# Autodesk Inventor assembly: MaquinaDeCorte
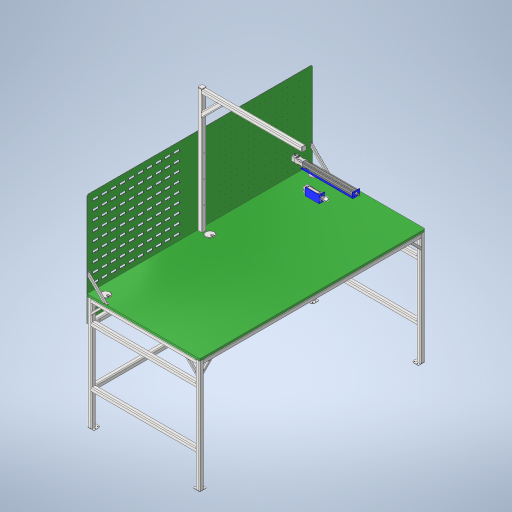
[picture p0: Inventor's stored thumbnail of the model, 512x512]
Saved by Autodesk Inventor 2023 (Build 270158000, 158)
## iProperties
Created: 2023-04-07
Part Number: MaquinaDeCorte
Document SubType Name: Assembly
Designer: Lenovo
Author: Lenovo
## Documents named in this file (6)
- D:\Esdek\Gemelo Digital\Corte de Tubos\MaquinaDeCorte.iam
- D:\Esdek\Gemelo Digital\Corte de Tubos\CADimportados\PistónElectromecánico\1470706 EPCO-25-300-3P-ST-E---(0).iam
- D:\Esdek\Gemelo Digital\Corte de Tubos\SoporteElectromecánico.ipt
- D:\Esdek\Gemelo Digital\Corte de Tubos\CADimportados\Main Table Assembly.ipt
- D:\Esdek\Gemelo Digital\Corte de Tubos\CADimportados\PistónHidráulico\163321 DNC-32-50-PPV---(asm_0).iam
- D:\Esdek\Gemelo Digital\Corte de Tubos\SoporteHidráhulicos.ipt
## Components (5 placed, 5 different names)
1. 1470706 EPCO-25-300-3P-ST-E---(0):1 [sub-assembly] — Mate:1, Mate:2, Mate:3
2. SoporteElectromecánico:1 — Mate:1, Mate:2, Mate:3
3. Main Table Assembly:1
4. 163321 DNC-32-50-PPV---(asm_0):1 [sub-assembly] — Mate:4, Mate:5, Mate:6
5. SoporteHidráhulicos:1 — Mate:4, Mate:5, Mate:6
## Relationships (6: Mate 6)
- Mate:1: 1470706 EPCO-25-300-3P-ST-E---(0):1 ↔ SoporteElectromecánico:1
- Mate:2: 1470706 EPCO-25-300-3P-ST-E---(0):1 ↔ SoporteElectromecánico:1
- Mate:3: 1470706 EPCO-25-300-3P-ST-E---(0):1 ↔ SoporteElectromecánico:1
- Mate:4: 163321 DNC-32-50-PPV---(asm_0):1 ↔ SoporteHidráhulicos:1
- Mate:5: 163321 DNC-32-50-PPV---(asm_0):1 ↔ SoporteHidráhulicos:1
- Mate:6: 163321 DNC-32-50-PPV---(asm_0):1 ↔ SoporteHidráhulicos:1
